# Autodesk Inventor assembly: Tool Rack Assembly
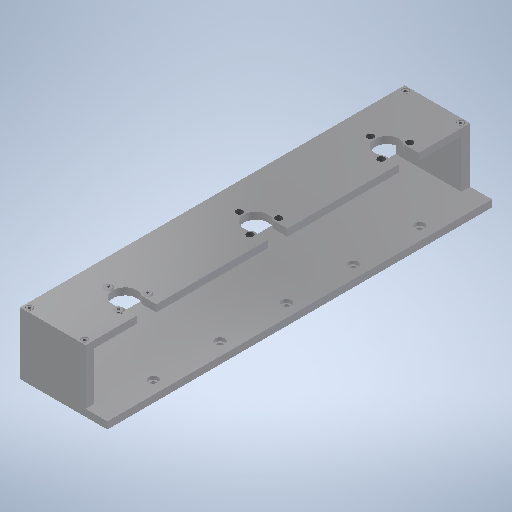
[picture p0: Inventor's stored thumbnail of the model, 512x512]
Saved by Autodesk Inventor 2025 (Build 290162000, 162)
## iProperties
Created: 2010-12-14
Part Number: Tool Rack Assembly
Document SubType Name: Assembly
Designer: berny
Author: berny
## Documents named in this file (6)
- C:\Users\cfang\Desktop\nebraska-silicon-lab\Hardware\General Gantry\Gantry Tool Rack\Tool Rack Assembly.iam
- C:\Users\cfang\Desktop\nebraska-silicon-lab\Hardware\General Gantry\Gantry Tool Rack\Bottom.ipt
- C:\Users\cfang\Desktop\nebraska-silicon-lab\Hardware\General Gantry\Gantry Tool Rack\Sides.ipt
- C:\Users\cfang\Desktop\nebraska-silicon-lab\Hardware\General Gantry\Gantry Tool Rack\Top.ipt
- C:\Users\cfang\Desktop\nebraska-silicon-lab\Hardware\General Gantry\Gantry Tool Rack\90128A212_Zinc-Plated Alloy Steel Socket Head Screw\90128A212_Zinc-Plated Alloy Steel Socket Head Screw.ipt
- C:\Users\cfang\Desktop\nebraska-silicon-lab\Hardware\General Gantry\Gantry Tool Rack\91375A617_Alloy Steel Cup-Point Set Screw\91375A617_Alloy Steel Cup-Point Set Screw.ipt
## Components (15 placed, 5 different names)
1. Top:1 — Flush:7, Flush:8, Mate:4, Insert:14, Insert:15, Insert:16, Insert:17, Insert:18, Insert:19, Insert:20
2. Sides:1 — Mate:2, Flush:3, Flush:4, Flush:7, Flush:8, Mate:4
3. Sides:2 — Mate:1, Mate:3, Flush:5, Flush:6
4. Bottom:1 — Mate:1, Mate:2, Flush:3, Flush:4, Mate:3, Flush:5, Flush:6, Insert:10, Insert:11, Insert:12, Insert:13
5. 90128A212_Zinc-Plated Alloy Steel Socket Head Screw:1 — Insert:10
6. 90128A212_Zinc-Plated Alloy Steel Socket Head Screw:2 — Insert:11
7. 90128A212_Zinc-Plated Alloy Steel Socket Head Screw:3 — Insert:12
8. 90128A212_Zinc-Plated Alloy Steel Socket Head Screw:4 — Insert:13
9. 90128A212_Zinc-Plated Alloy Steel Socket Head Screw:5 — Insert:17
10. 90128A212_Zinc-Plated Alloy Steel Socket Head Screw:6 — Insert:16
11. 90128A212_Zinc-Plated Alloy Steel Socket Head Screw:7 — Insert:15
12. 90128A212_Zinc-Plated Alloy Steel Socket Head Screw:8 — Insert:14
13. 91375A617_Alloy Steel Cup-Point Set Screw:1 — Insert:18
14. 91375A617_Alloy Steel Cup-Point Set Screw:2 — Insert:19
15. 91375A617_Alloy Steel Cup-Point Set Screw:3 — Insert:20
## Relationships (21: Insert 11, Flush 6, Mate 4)
- Mate:1: Sides:2 ↔ Bottom:1
- Mate:2: Sides:1 ↔ Bottom:1
- Flush:3: Sides:1 ↔ Bottom:1
- Flush:4: Sides:1 ↔ Bottom:1
- Mate:3: Sides:2 ↔ Bottom:1
- Flush:5: Sides:2 ↔ Bottom:1
- Flush:6: Sides:2 ↔ Bottom:1
- Flush:7: Top:1 ↔ Sides:1
- Flush:8: Top:1 ↔ Sides:1
- Mate:4: Top:1 ↔ Sides:1
- Insert:10: Bottom:1 ↔ 90128A212_Zinc-Plated Alloy Steel Socket Head Screw:1
- Insert:11: Bottom:1 ↔ 90128A212_Zinc-Plated Alloy Steel Socket Head Screw:2
- Insert:12: Bottom:1 ↔ 90128A212_Zinc-Plated Alloy Steel Socket Head Screw:3
- Insert:13: Bottom:1 ↔ 90128A212_Zinc-Plated Alloy Steel Socket Head Screw:4
- Insert:14: Top:1 ↔ 90128A212_Zinc-Plated Alloy Steel Socket Head Screw:8
- Insert:15: Top:1 ↔ 90128A212_Zinc-Plated Alloy Steel Socket Head Screw:7
- Insert:16: Top:1 ↔ 90128A212_Zinc-Plated Alloy Steel Socket Head Screw:6
- Insert:17: Top:1 ↔ 90128A212_Zinc-Plated Alloy Steel Socket Head Screw:5
- Insert:18 (2.5 mm): Top:1 ↔ 91375A617_Alloy Steel Cup-Point Set Screw:1
- Insert:19 (2.5 mm): Top:1 ↔ 91375A617_Alloy Steel Cup-Point Set Screw:2
- Insert:20 (2.5 mm): Top:1 ↔ 91375A617_Alloy Steel Cup-Point Set Screw:3
